# Autodesk Inventor assembly: Hand
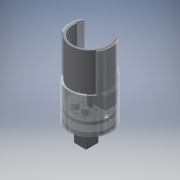
[picture p0: Inventor's stored thumbnail of the model, 180x180]
Saved by Autodesk Inventor 2016 (Build 200138000, 138)
## iProperties
Created: 2016-11-13
Part Number: Hand
Material: 一般
Document SubType Name: Assembly
Designer: Daisuke
Author: Daisuke
## Documents named in this file (10)
- C:\Users\Daisuke\Documents\GitHub\CAD\Hand\ver2\Hand.iam
- C:\Users\Daisuke\Documents\GitHub\CAD\Hand\ver2\outsideCover.iam
- C:\Users\Daisuke\Documents\GitHub\CAD\Hand\ver2\Servo.iam
- C:\Users\Daisuke\Documents\GitHub\CAD\Hand\ver2\outsideBottom2.ipt
- C:\Users\Daisuke\Documents\GitHub\CAD\Hand\ver2\outsideBottom1.ipt
- C:\Users\Daisuke\Documents\GitHub\CAD\Hand\ver2\Servo.ipt
- C:\Users\Daisuke\Documents\GitHub\CAD\Hand\ver2\ServoArm.ipt
- C:\Users\Daisuke\Documents\GitHub\CAD\Hand\ver2\UFL08 -Housing.ipt
- C:\Users\Daisuke\Documents\GitHub\CAD\Hand\ver2\UltrasonicDistanceSencor.ipt
- C:\Users\Daisuke\Documents\GitHub\CAD\Hand\ver2\insideHand.iam
## Components (9 placed, 8 different names)
1. outsideCover:1 [sub-assembly] — メイト:1, メイト:2, 挿入:13, 挿入:14
2. Servo:1 [sub-assembly] — 挿入:1, 挿入:2, 挿入:3
3. outsideBottom2:1 — 挿入:9, 挿入:10, 挿入:11, メイト:2, 挿入:14
4. outsideBottom1:1 — 挿入:1, 挿入:2, 挿入:3, 挿入:4, 挿入:5, 挿入:6, 挿入:7, メイト:1
5. Servo:2 — 挿入:8
6. ServoArm:1 — 挿入:8, 挿入:9, 挿入:10, 挿入:11
7. UFL08 -Housing:1 — 挿入:6, 挿入:7, 挿入:12
8. UltrasonicDistanceSencor:1 — 挿入:4, 挿入:5
9. insideHand:1 [sub-assembly] — 挿入:12, 挿入:13
## Relationships (16: Insert 14, Mate 2)
- 挿入:1 [Insert]: Servo:1 ↔ outsideBottom1:1
- 挿入:2 [Insert]: Servo:1 ↔ outsideBottom1:1
- 挿入:3 [Insert]: Servo:1 ↔ outsideBottom1:1
- 挿入:4 [Insert]: outsideBottom1:1 ↔ UltrasonicDistanceSencor:1
- 挿入:5 [Insert]: outsideBottom1:1 ↔ UltrasonicDistanceSencor:1
- 挿入:6 [Insert]: outsideBottom1:1 ↔ UFL08 -Housing:1
- 挿入:7 [Insert]: outsideBottom1:1 ↔ UFL08 -Housing:1
- 挿入:8 [Insert] (0.5 mm): Servo:2 ↔ ServoArm:1
- 挿入:9 [Insert]: outsideBottom2:1 ↔ ServoArm:1
- 挿入:10 [Insert]: outsideBottom2:1 ↔ ServoArm:1
- 挿入:11 [Insert]: outsideBottom2:1 ↔ ServoArm:1
- 挿入:12 [Insert]: UFL08 -Housing:1 ↔ insideHand:1
- メイト:1 [Mate]: outsideCover:1 ↔ outsideBottom1:1
- メイト:2 [Mate]: outsideCover:1 ↔ outsideBottom2:1
- 挿入:13 [Insert]: outsideCover:1 ↔ insideHand:1
- 挿入:14 [Insert]: outsideCover:1 ↔ outsideBottom2:1
